# Autodesk Inventor assembly: Sklop
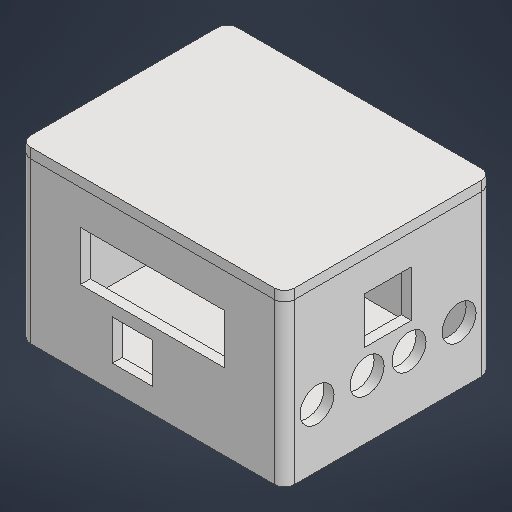
[picture p0: Inventor's stored thumbnail of the model, 512x512]
Saved by Autodesk Inventor 2025.2 (Build 292293000, 293)
## iProperties
Created: 2024-12-17
Part Number: Sklop
Document SubType Name: Assembly
Designer: antem
Author: antem
## Documents named in this file (8)
- C:\Users\antem\Desktop\Naks\Sklop.iam
- C:\Users\antem\Desktop\Naks\kucisteDonji.ipt
- C:\Users\antem\Desktop\Naks\rasberry.ipt
- C:\Users\antem\Desktop\Naks\plocica.ipt
- C:\Users\antem\Desktop\Naks\ultrasonic.ipt
- C:\Users\antem\Desktop\Naks\pir.ipt
- C:\Users\antem\Desktop\Naks\display.ipt
- C:\Users\antem\Desktop\Naks\kucisteGornji.ipt
## Components (8 placed, 7 different names)
1. kucisteDonji:1 — Mate:1, Mate:2, Mate:3, Mate:4, Angle:1, Mate:5, Mate:7, Mate:8, Mate:9
2. rasberry:1 — Mate:1, Angle:1
3. plocica:1 — Mate:5, Angle:2
4. ultrasonic:1 — Flush:1, Flush:2, Angle:2
5. ultrasonic:2 — Flush:1, Flush:2, Mate:7
6. pir:1 — Mate:6, Angle:3, Mate:8
7. display:1 — Mate:9
8. kucisteGornji:1 — Mate:10, Flush:3
## Relationships (16: Mate 10, Angle 3, Flush 3)
- Mate:1: kucisteDonji:1 ↔ rasberry:1
- Mate:2: kucisteDonji:1
- Mate:3: kucisteDonji:1
- Mate:4: kucisteDonji:1
- Angle:1 (180 deg): kucisteDonji:1 ↔ rasberry:1
- Mate:5: kucisteDonji:1 ↔ plocica:1
- Flush:1: ultrasonic:1 ↔ ultrasonic:2
- Flush:2: ultrasonic:1 ↔ ultrasonic:2
- Angle:2 (0 deg): plocica:1 ↔ ultrasonic:1
- Mate:6: pir:1
- Angle:3 (0 deg): pir:1
- Mate:7: kucisteDonji:1 ↔ ultrasonic:2
- Mate:8: kucisteDonji:1 ↔ pir:1
- Mate:9: kucisteDonji:1 ↔ display:1
- Mate:10: kucisteGornji:1
- Flush:3: kucisteGornji:1
